# Autodesk Inventor assembly: 2021-2022 Arm Base
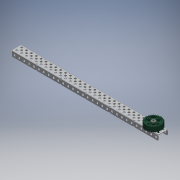
[picture p0: Inventor's stored thumbnail of the model, 180x180]
Saved by Autodesk Inventor 2019 (Build 230136000, 136)
## iProperties
Created: 2021-09-09
Part Number: 2021-2022 Arm Base
Document SubType Name: Assembly
Designer: 22spencen
Author: 22spencen
## Documents named in this file (5)
- \\Chopper\2022\22spencen\Documents\VEX_CAD\Assemblies\2021-2022 Arm Base.iam
- \\Chopper\2022\22spencen\Documents\VEX_CAD\Part Files\VEX Parts Library 2016\Imperial\Structure\C-Channel 1x2x1x30 Hole.ipt
- \\Chopper\2022\22spencen\Documents\VEX_CAD\Part Files\VEX Parts Library 2016\Imperial\Motion\Bearing Flat.ipt
- \\Chopper\2022\22spencen\Documents\VEX_CAD\Part Files\VEX Parts Library 2016\Imperial\Motion\Gears\High Strength 36 Tooth Gear.ipt
- \\Chopper\2022\22spencen\Documents\VEX_CAD\Part Files\VEX Parts Library 2016\Imperial\Motion\Metal_Shaft_Inserts_276-3881-002.ipt
## Components (5 placed, 4 different names)
1. C-Channel 1x2x1x30 Hole:1 — Mate:1, Mate:7
2. Bearing Flat:1 — Mate:1
3. High Strength 36 Tooth Gear:1 — Mate:2, Mate:3, Mate:4, Mate:5, Mate:6, Mate:7
4. Metal_Shaft_Inserts_276-3881-002:1 — Mate:2, Mate:3, Mate:4, Flush:1
5. Metal_Shaft_Inserts_276-3881-002:2 — Mate:5, Mate:6, Flush:1
## Relationships (8: Mate 7, Flush 1)
- Mate:1: C-Channel 1x2x1x30 Hole:1 ↔ Bearing Flat:1
- Mate:2: High Strength 36 Tooth Gear:1 ↔ Metal_Shaft_Inserts_276-3881-002:1
- Mate:3: High Strength 36 Tooth Gear:1 ↔ Metal_Shaft_Inserts_276-3881-002:1
- Mate:4: High Strength 36 Tooth Gear:1 ↔ Metal_Shaft_Inserts_276-3881-002:1
- Mate:5: High Strength 36 Tooth Gear:1 ↔ Metal_Shaft_Inserts_276-3881-002:2
- Mate:6: High Strength 36 Tooth Gear:1 ↔ Metal_Shaft_Inserts_276-3881-002:2
- Flush:1: Metal_Shaft_Inserts_276-3881-002:1 ↔ Metal_Shaft_Inserts_276-3881-002:2
- Mate:7: C-Channel 1x2x1x30 Hole:1 ↔ High Strength 36 Tooth Gear:1
